# Autodesk Inventor assembly: Visual Assembly
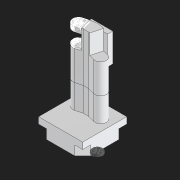
[picture p0: Inventor's stored thumbnail of the model, 180x180]
Saved by Autodesk Inventor 2017 SP1 (Build 210196100, 196)
## iProperties
Created: 2018-03-03
Part Number: Visual Assembly
Document SubType Name: Assembly
Designer: Zach
Author: Zach
## Documents named in this file (5)
- C:\Users\Zach\Documents\GitHub\tr1_description\meshes\Visual Assembly\Visual Assembly.iam
- C:\Users\Zach\Documents\GitHub\tr1_description\meshes\Visual Assembly\Base.ipt
- C:\Users\Zach\Documents\GitHub\tr1_description\meshes\Visual Assembly\Body.ipt
- C:\Users\Zach\Documents\GitHub\tr1_description\meshes\Visual Assembly\Wheel.ipt
- C:\Users\Zach\Documents\GitHub\tr1_description\meshes\Visual Assembly\Arm1.iam
## Components (4 placed, 4 different names)
1. Base:1 — Mate:1, Mate:2, Mate:3
2. Body:1 — Mate:1, Mate:2, Mate:3, Mate:4, Mate:5, Mate:6
3. Wheel:1
4. Arm1:1 [sub-assembly] — Mate:4, Mate:5, Mate:6
## Relationships (6: Mate 6)
- Mate:1: Base:1 ↔ Body:1
- Mate:2: Base:1 ↔ Body:1
- Mate:3: Base:1 ↔ Body:1
- Mate:4: Body:1 ↔ Arm1:1
- Mate:5: Body:1 ↔ Arm1:1
- Mate:6: Body:1 ↔ Arm1:1
